# Autodesk Inventor assembly: Assembly2
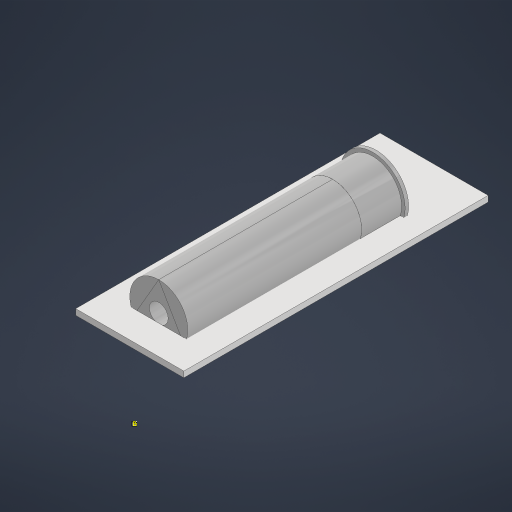
[picture p0: Inventor's stored thumbnail of the model, 512x512]
Saved by Autodesk Inventor 2024.3 (Build 283343000, 343)
## iProperties
Created: 2025-08-18
Part Number: Assembly2
Document SubType Name: Assembly
Designer: giuseppe
Author: giuseppe
## Documents named in this file (3)
- C:\Users\giuseppe\Desktop\Buckshot-Ruolette\CAD\mostra cartucce\V2\Assembly2.iam
- C:\Users\giuseppe\Desktop\Buckshot-Ruolette\CAD\mostra cartucce\rotater shell v3.ipt
- C:\Users\giuseppe\Desktop\Buckshot-Ruolette\CAD\mostra cartucce\V2\holderV2.ipt
## Components (2 placed, 2 different names)
1. rotater shell v3:1 — Flush:1, Flush:2
2. holderV2:1 — Flush:1, Flush:2
## Relationships (2: Flush 2)
- Flush:1: rotater shell v3:1 ↔ holderV2:1
- Flush:2: rotater shell v3:1 ↔ holderV2:1
